# Autodesk Inventor assembly: Arm Lower Shortened
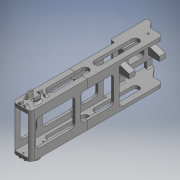
[picture p0: Inventor's stored thumbnail of the model, 180x180]
Saved by Autodesk Inventor 2020.5 (Build 245400000, 400)
## iProperties
Created: 2023-03-26
Part Number: Arm Lower Shortened
Document SubType Name: Assembly
Designer: Wes
Author: Wes
## Documents named in this file (3)
- C:\Users\Wes\Documents\Wes Stuff\Programming\Python\CPEN291\P2_L2B_G8\3D Design\Arm Lower Shortened.iam
- C:\Users\Wes\Documents\Wes Stuff\Programming\Python\CPEN291\P2_L2B_G8\3D Design\Arm Lower Bottom.ipt
- C:\Users\Wes\Documents\Wes Stuff\Programming\Python\CPEN291\P2_L2B_G8\3D Design\Arm Lower Top.ipt
## Components (2 placed, 2 different names)
1. Arm Lower Bottom:1 — Flush:1, Flush:2, Mate:1
2. Arm Lower Top:1 — Flush:1, Flush:2, Mate:1
## Relationships (3: Flush 2, Mate 1)
- Flush:1: Arm Lower Bottom:1 ↔ Arm Lower Top:1
- Flush:2: Arm Lower Bottom:1 ↔ Arm Lower Top:1
- Mate:1: Arm Lower Bottom:1 ↔ Arm Lower Top:1
